# Autodesk Inventor assembly: fINAL Assembly
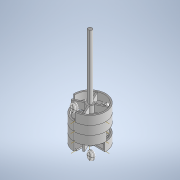
[picture p0: Inventor's stored thumbnail of the model, 180x180]
Saved by Autodesk Inventor 2022 (Build 260153000, 153)
## iProperties
Created: 2022-03-07
Part Number: fINAL Assembly
Document SubType Name: Assembly
Designer: Alicia
Author: Alicia
## Documents named in this file (8)
- C:\Users\Public\Documents\Autodesk\Inventor 2022\Dispenser\Plan B Design\fINAL Assembly.iam
- C:\Users\Public\Documents\Autodesk\Inventor 2022\Dispenser\Plan B Design\base layer 1.ipt
- C:\Users\Public\Documents\Autodesk\Inventor 2022\Dispenser\Plan B Design\wheel of the walls.ipt
- C:\Users\Public\Documents\Autodesk\Inventor 2022\Dispenser\Plan B Design\shaft.ipt
- C:\Users\Public\Documents\Autodesk\Inventor 2022\Dispenser\Plan B Design\base layer 2.ipt
- C:\Users\Public\Documents\Autodesk\Inventor 2022\Dispenser\Plan B Design\base layer 3.ipt
- C:\Users\Public\Documents\Autodesk\Inventor 2022\Dispenser\Plan B Design\base layer 4.ipt
- C:\Users\Public\Documents\Autodesk\Inventor 2022\Dispenser\Plan B Design\pill.ipt
## Components (14 placed, 7 different names)
1. base layer 1:1 — Mate:1, Mate:2, Insert:1, Mate:4, Flush:1, Mate:6
2. wheel of the walls:1 — Insert:1, Insert:2, Mate:3
3. shaft:1 — Insert:2, Mate:3, Mate:5, Mate:8, Mate:10
4. base layer 2:1 — Mate:4, Flush:1, Insert:3, Mate:6, Mate:7, Flush:2
5. wheel of the walls:2 — Insert:3, Mate:5
6. base layer 3:1 — Mate:7, Flush:2, Insert:4, Mate:9, Flush:3
7. wheel of the walls:3 — Mate:8, Insert:4
8. base layer 4:1 — Mate:9, Insert:5, Flush:3, Mate:11, Mate:12
9. wheel of the walls:4 — Mate:10, Insert:5
10. pill:1 — Mate:12
11. pill:2 — Mate:11
12. pill:5
13. pill:6
14. pill:7
## Relationships (20: Mate 12, Insert 5, Flush 3)
- Mate:1: base layer 1:1
- Mate:2: base layer 1:1
- Insert:1 (2 mm): base layer 1:1 ↔ wheel of the walls:1
- Insert:2: wheel of the walls:1 ↔ shaft:1
- Mate:3: wheel of the walls:1 ↔ shaft:1
- Mate:4: base layer 1:1 ↔ base layer 2:1
- Flush:1: base layer 1:1 ↔ base layer 2:1
- Insert:3 (-2 mm): base layer 2:1 ↔ wheel of the walls:2
- Mate:5: shaft:1 ↔ wheel of the walls:2
- Mate:6: base layer 1:1 ↔ base layer 2:1
- Mate:7: base layer 2:1 ↔ base layer 3:1
- Flush:2: base layer 2:1 ↔ base layer 3:1
- Mate:8: shaft:1 ↔ wheel of the walls:3
- Insert:4: base layer 3:1 ↔ wheel of the walls:3
- Mate:9: base layer 3:1 ↔ base layer 4:1
- Mate:10: shaft:1 ↔ wheel of the walls:4
- Insert:5: base layer 4:1 ↔ wheel of the walls:4
- Flush:3: base layer 3:1 ↔ base layer 4:1
- Mate:11: base layer 4:1 ↔ pill:2
- Mate:12: base layer 4:1 ↔ pill:1
